# Autodesk Inventor assembly: Motor
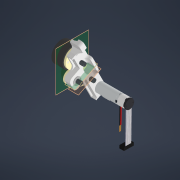
[picture p0: Inventor's stored thumbnail of the model, 180x180]
Saved by Autodesk Inventor 2022 (Build 260153000, 153)
## iProperties
Created: 2021-09-24
Part Number: Motor
Document SubType Name: Assembly
Designer: shiok
Mass: 24.8351 g
Surface Area: 226.347 cm^2
Volume: 18.047 cm^3
Density: 1.37613 g/cm^3
Author: shiok
## Documents named in this file (8)
- C:\Users\shiok\Documents\GitHub\murakumo\inventor\Motor.iam
- C:\Users\shiok\Documents\GitHub\murakumo\inventor\maxon DCX 10L.iam
- C:\Users\shiok\Documents\GitHub\murakumo\inventor\Tire.iam
- C:\Users\shiok\Documents\GitHub\murakumo\inventor\piniongear_41_middle.ipt
- C:\Users\shiok\Documents\GitHub\murakumo\inventor\piniongear_41_src.ipt
- C:\Users\shiok\Documents\GitHub\murakumo\inventor\shaft_short.ipt
- C:\Users\shiok\Documents\GitHub\murakumo\inventor\MotorBracketv2.ipt
- C:\Users\shiok\Documents\GitHub\murakumo\inventor\FL674ZZ_MIR.ipt
## Components (9 placed, 7 different names)
1. Tire:1 [sub-assembly] — メイト:6, フラッシュ:1, メイト:11, 対称度:1
2. MotorBracketv2:1 — メイト:1, メイト:2, メイト:3, メイト:4, メイト:6, メイト:7, メイト:8, メイト:10, メイト:11
3. Tire:2 [sub-assembly] — メイト:7, フラッシュ:1, フラッシュ:2, フラッシュ:3, 対称度:1
4. maxon DCX 10L:1 [sub-assembly] — メイト:8, メイト:9, メイト:10
5. FL674ZZ_MIR:1 — メイト:3, メイト:4
6. FL674ZZ_MIR:2 — メイト:1, メイト:2, メイト:5
7. piniongear_41_middle:1 — 挿入:6, フラッシュ:2
8. piniongear_41_src:1 — フラッシュ:3, メイト:9
9. shaft_short:1 — 挿入:6, メイト:5
## Relationships (16: Mate 11, Flush 3, Insert 1, Symmetry 1)
- 挿入:6 [Insert]: piniongear_41_middle:1 ↔ shaft_short:1
- メイト:1 [Mate]: MotorBracketv2:1 ↔ FL674ZZ_MIR:2
- メイト:2 [Mate]: MotorBracketv2:1 ↔ FL674ZZ_MIR:2
- メイト:3 [Mate]: MotorBracketv2:1 ↔ FL674ZZ_MIR:1
- メイト:4 [Mate]: MotorBracketv2:1 ↔ FL674ZZ_MIR:1
- メイト:5 [Mate]: FL674ZZ_MIR:2 ↔ shaft_short:1
- メイト:6 [Mate]: Tire:1 ↔ MotorBracketv2:1
- メイト:7 [Mate]: MotorBracketv2:1 ↔ Tire:2
- フラッシュ:1 [Flush]: Tire:1 ↔ Tire:2
- フラッシュ:2 [Flush]: Tire:2 ↔ piniongear_41_middle:1
- フラッシュ:3 [Flush]: Tire:2 ↔ piniongear_41_src:1
- メイト:8 [Mate]: MotorBracketv2:1 ↔ maxon DCX 10L:1
- メイト:9 [Mate]: maxon DCX 10L:1 ↔ piniongear_41_src:1
- メイト:10 [Mate]: MotorBracketv2:1 ↔ maxon DCX 10L:1
- メイト:11 [Mate] (1 mm): Tire:1 ↔ MotorBracketv2:1
- 対称度:1 [Symmetry]: Tire:1 ↔ Tire:2
